# Autodesk Inventor assembly: fight_robot
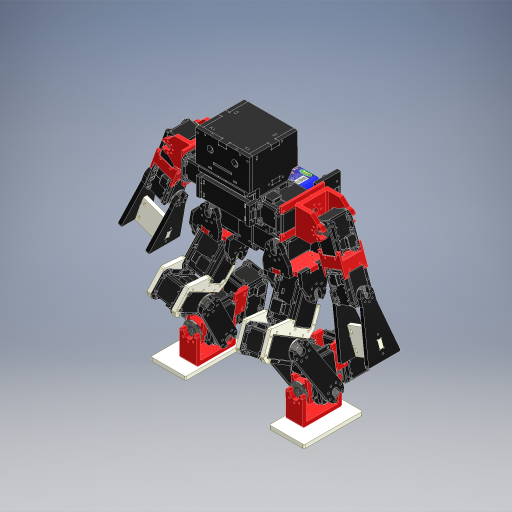
[picture p0: Inventor's stored thumbnail of the model, 512x512]
Saved by Autodesk Inventor 2024 (Build 280153000, 153)
## iProperties
Created: 2024-09-15
Part Number: fight_robot
Document SubType Name: Assembly
Designer: msi
Author: msi
## Documents named in this file (9)
- C:\Users\msi\GITHUB\19th_intern_kgh_fight_robot\부품\fight_robot.iam
- C:\Users\msi\GITHUB\19th_intern_kgh_fight_robot\부품\Upper_body\Body\body.iam
- C:\Users\msi\GITHUB\19th_intern_kgh_fight_robot\부품\Upper_body\Arm\arm_left.iam
- C:\Users\msi\GITHUB\19th_intern_kgh_fight_robot\부품\Lower_Body\Hip_joint\hip_joint.iam
- C:\Users\msi\GITHUB\19th_intern_kgh_fight_robot\부품\Lower_Body\Thigh\thigh_left.iam
- C:\Users\msi\GITHUB\19th_intern_kgh_fight_robot\부품\Lower_Body\Thigh\thigh_right.iam
- C:\Users\msi\GITHUB\19th_intern_kgh_fight_robot\부품\Lower_Body\Calf\calf_left.iam
- C:\Users\msi\GITHUB\19th_intern_kgh_fight_robot\부품\Lower_Body\Calf\calf_right.iam
- C:\Users\msi\GITHUB\19th_intern_kgh_fight_robot\부품\Upper_body\Arm\arm_right.iam
## Components (8 placed, 8 different names)
1. body:1 [sub-assembly] — 삽입:1, 삽입:2, 삽입:9, 삽입:10, 삽입:11, 삽입:12
2. hip_joint:1 [sub-assembly] — 삽입:1, 삽입:2, 삽입:3, 삽입:4, 삽입:5, 삽입:6
3. thigh_right:1 [sub-assembly] — 삽입:3, 삽입:4, 삽입:7, 각도:2
4. thigh_left:1 [sub-assembly] — 삽입:5, 삽입:6, 삽입:8, 각도:1
5. calf_left:1 [sub-assembly] — 삽입:8, 각도:1
6. calf_right:1 [sub-assembly] — 삽입:7, 각도:2
7. arm_left:1 [sub-assembly] — 삽입:9, 삽입:10
8. arm_right:1 [sub-assembly] — 삽입:11, 삽입:12
## Relationships (14: Insert 12, Angle 2)
- 삽입:1 [Insert]: body:1 ↔ hip_joint:1
- 삽입:2 [Insert]: body:1 ↔ hip_joint:1
- 삽입:3 [Insert]: hip_joint:1 ↔ thigh_right:1
- 삽입:4 [Insert]: hip_joint:1 ↔ thigh_right:1
- 삽입:5 [Insert]: hip_joint:1 ↔ thigh_left:1
- 삽입:6 [Insert]: hip_joint:1 ↔ thigh_left:1
- 삽입:7 [Insert]: thigh_right:1 ↔ calf_right:1
- 삽입:8 [Insert]: thigh_left:1 ↔ calf_left:1
- 각도:1 [Angle] (30 deg): thigh_left:1 ↔ calf_left:1
- 각도:2 [Angle] (-30 deg): thigh_right:1 ↔ calf_right:1
- 삽입:9 [Insert]: body:1 ↔ arm_left:1
- 삽입:10 [Insert]: body:1 ↔ arm_left:1
- 삽입:11 [Insert]: body:1 ↔ arm_right:1
- 삽입:12 [Insert]: body:1 ↔ arm_right:1
